# Autodesk Inventor assembly: Roller
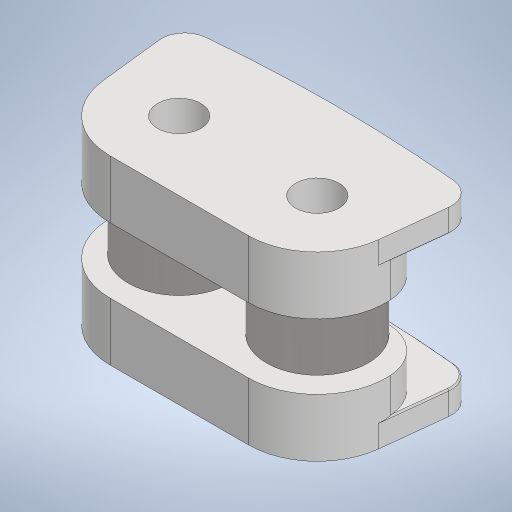
[picture p0: Inventor's stored thumbnail of the model, 512x512]
Saved by Autodesk Inventor 2023.4 (Build 274418000, 418)
## iProperties
Created: 2024-04-30
Part Number: Roller
Document SubType Name: Assembly
Designer: Nathan Cai
Author: Nathan Cai
## Documents named in this file (3)
- E:\Documents\Inventor\Reaction Ring V0.1\Roller.iam
- E:\Documents\Inventor\Reaction Ring V0.1\Thrust Bushing.ipt
- E:\Documents\Inventor\Reaction Ring V0.1\BB 3x7x3 - Copy.ipt
## Components (4 placed, 2 different names)
1. Thrust Bushing:1 — Mate:1, Mate:2, Mate:3
2. BB 3x7x3 - Copy:1 — Mate:1, Mate:3, Flush:1, Mate:4, Mate:6
3. BB 3x7x3 - Copy:2 — Mate:2, Flush:1, Mate:5
4. Thrust Bushing:2 — Mate:4, Mate:5, Mate:6
## Relationships (7: Mate 6, Flush 1)
- Mate:1: Thrust Bushing:1 ↔ BB 3x7x3 - Copy:1
- Mate:2: Thrust Bushing:1 ↔ BB 3x7x3 - Copy:2
- Mate:3 (0.25 mm): Thrust Bushing:1 ↔ BB 3x7x3 - Copy:1
- Flush:1: BB 3x7x3 - Copy:1 ↔ BB 3x7x3 - Copy:2
- Mate:4 (0.25 mm): BB 3x7x3 - Copy:1 ↔ Thrust Bushing:2
- Mate:5: BB 3x7x3 - Copy:2 ↔ Thrust Bushing:2
- Mate:6: BB 3x7x3 - Copy:1 ↔ Thrust Bushing:2
